# Autodesk Inventor assembly: Eingebaute Elektronik
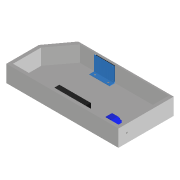
[picture p0: Inventor's stored thumbnail of the model, 180x180]
Saved by Autodesk Inventor 2020 (Build 240168000, 168)
## iProperties
Created: 2022-03-17
Part Number: Eingebaute Elektronik
Document SubType Name: Assembly
Designer: Mike
Author: Mike
## Documents named in this file (11)
- C:\Users\Mike\Desktop\Digitales Inhaltsverzeichnis\Eingebaute Elektronik.iam
- C:\Users\Mike\Desktop\Digitales Inhaltsverzeichnis\Elektronik\Armlehne Dummy.ipt
- C:\Users\Mike\Desktop\Digitales Inhaltsverzeichnis\Elektronik\Hutschiene.ipt
- C:\Users\Mike\Desktop\Digitales Inhaltsverzeichnis\Elektronik\Netztransformator.ipt
- C:\Users\Mike\Desktop\Digitales Inhaltsverzeichnis\Elektronik\Netzteil.ipt
- C:\Users\Mike\Desktop\Digitales Inhaltsverzeichnis\Elektronik\Handy Ablage.ipt
- C:\Users\Mike\Desktop\Digitales Inhaltsverzeichnis\Elektronik\Halterung Platine.ipt
- C:\Users\Mike\Desktop\Digitales Inhaltsverzeichnis\Elektronik\Platine Dummy.ipt
- C:\Users\Mike\Documents\Inventor\Content Center Files\R2020\de-DE\AS 1427(07)\AS 1427 - M3 x 5(6) II.ipt
- C:\Users\Mike\Documents\Inventor\Content Center Files\R2020\de-DE\AS 1427(07)\AS 1427 - M5 x 8(6) II.ipt
- C:\Users\Mike\Documents\Inventor\Content Center Files\R2020\de-DE\AS 1427(07)\AS 1427 - M3 x 8(6) II.ipt
## Components (17 placed, 10 different names)
1. Armlehne Dummy:1 — Passend:1, Passend:2, Passend:3, Passend:6, Fluchtend:2, Passend:7, Passend:8, Passend:9, Fluchtend:3, Passend:10, Passend:12, Passend:13
2. Hutschiene:1 — Passend:1, Passend:2, Passend:3, Passend:4, Passend:5, Fluchtend:1, Einfügen:9, Einfügen:10
3. Netztransformator:1 — Passend:4, Passend:5, Fluchtend:1
4. Netzteil:1 — Passend:6, Fluchtend:2, Passend:7, Einfügen:11, Einfügen:12
5. Handy Ablage:1 — Passend:8, Passend:9, Fluchtend:3
6. Halterung Platine:1 — Passend:10, Passend:11, Einfügen:1, Einfügen:2, Passend:12, Passend:13, Einfügen:7, Einfügen:8
7. Platine Dummy:1 — Passend:11, Einfügen:1, Einfügen:2, Einfügen:3, Einfügen:4, Einfügen:5, Einfügen:6
8. AS 1427 Z - Metrisch M3 x 5:1 — Einfügen:3
9. AS 1427 Z - Metrisch M3 x 5:2 — Einfügen:4
10. AS 1427 Z - Metrisch M3 x 5:3 — Einfügen:5
11. AS 1427 Z - Metrisch M3 x 5:4 — Einfügen:6
12. AS 1427 Z - Metrisch M5 x 8:1 — Einfügen:8
13. AS 1427 Z - Metrisch M5 x 8:2 — Einfügen:7
14. AS 1427 Z - Metrisch M3 x 8:1 — Einfügen:9
15. AS 1427 Z - Metrisch M3 x 8:2 — Einfügen:10
16. AS 1427 Z - Metrisch M3 x 5:5 — Einfügen:11
17. AS 1427 Z - Metrisch M3 x 5:6 — Einfügen:12
## Relationships (28: Mate 13, Insert 12, Flush 3)
- Passend:1 [Mate]: Armlehne Dummy:1 ↔ Hutschiene:1
- Passend:2 [Mate] (50 mm): Armlehne Dummy:1 ↔ Hutschiene:1
- Passend:3 [Mate] (50 mm): Armlehne Dummy:1 ↔ Hutschiene:1
- Passend:4 [Mate]: Hutschiene:1 ↔ Netztransformator:1
- Passend:5 [Mate]: Hutschiene:1 ↔ Netztransformator:1
- Fluchtend:1 [Flush] (30 mm): Hutschiene:1 ↔ Netztransformator:1
- Passend:6 [Mate]: Armlehne Dummy:1 ↔ Netzteil:1
- Fluchtend:2 [Flush] (5 mm): Armlehne Dummy:1 ↔ Netzteil:1
- Passend:7 [Mate] (200 mm): Armlehne Dummy:1 ↔ Netzteil:1
- Passend:8 [Mate]: Armlehne Dummy:1 ↔ Handy Ablage:1
- Passend:9 [Mate]: Armlehne Dummy:1 ↔ Handy Ablage:1
- Fluchtend:3 [Flush] (2 mm): Armlehne Dummy:1 ↔ Handy Ablage:1
- Passend:10 [Mate]: Armlehne Dummy:1 ↔ Halterung Platine:1
- Passend:11 [Mate]: Halterung Platine:1 ↔ Platine Dummy:1
- Einfügen:1 [Insert]: Halterung Platine:1 ↔ Platine Dummy:1
- Einfügen:2 [Insert]: Halterung Platine:1 ↔ Platine Dummy:1
- Einfügen:3 [Insert]: Platine Dummy:1 ↔ AS 1427 Z - Metrisch M3 x 5:1
- Einfügen:4 [Insert]: Platine Dummy:1 ↔ AS 1427 Z - Metrisch M3 x 5:2
- Einfügen:5 [Insert]: Platine Dummy:1 ↔ AS 1427 Z - Metrisch M3 x 5:3
- Einfügen:6 [Insert]: Platine Dummy:1 ↔ AS 1427 Z - Metrisch M3 x 5:4
- Passend:12 [Mate] (3 mm): Armlehne Dummy:1 ↔ Halterung Platine:1
- Passend:13 [Mate]: Armlehne Dummy:1 ↔ Halterung Platine:1
- Einfügen:7 [Insert]: Halterung Platine:1 ↔ AS 1427 Z - Metrisch M5 x 8:2
- Einfügen:8 [Insert]: Halterung Platine:1 ↔ AS 1427 Z - Metrisch M5 x 8:1
- Einfügen:9 [Insert]: Hutschiene:1 ↔ AS 1427 Z - Metrisch M3 x 8:1
- Einfügen:10 [Insert]: Hutschiene:1 ↔ AS 1427 Z - Metrisch M3 x 8:2
- Einfügen:11 [Insert]: Netzteil:1 ↔ AS 1427 Z - Metrisch M3 x 5:5
- Einfügen:12 [Insert]: Netzteil:1 ↔ AS 1427 Z - Metrisch M3 x 5:6
